# Autodesk Inventor assembly: Pick_&_Place_Nozzle_Assembly
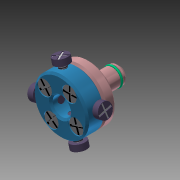
[picture p0: Inventor's stored thumbnail of the model, 180x180]
Saved by Autodesk Inventor 2015 (Build 190159000, 159)
## iProperties
Created: 2015-01-06
Part Number: Pick_&_Place_Nozzle_Assembly
Document SubType Name: Assembly
Designer: ice
Author: ice
## Documents named in this file (8)
- C:\Users\ice\Documents\GitHub\PnP-Magnetic-Tool-Tip\Inventor\Magnetic_Extender_Assembly.iam
- C:\Users\ice\Documents\GitHub\PnP-Magnetic-Tool-Tip\Inventor\Magnet_Extender_Split_Top.ipt
- C:\Users\ice\Documents\GitHub\PnP-Magnetic-Tool-Tip\Inventor\Magnet_Extender_Split_Bottom.ipt
- C:\Users\ice\Documents\GitHub\PnP-Magnetic-Tool-Tip\Inventor\M2x5_D963.ipt
- C:\Users\ice\Documents\GitHub\PnP-Magnetic-Tool-Tip\Inventor\o_ring_3.18_0.5.ipt
- C:\Users\ice\Documents\GitHub\PnP-Magnetic-Tool-Tip\Inventor\M2x5_D85_PANHD.ipt
- C:\Users\ice\Documents\GitHub\PnP-Magnetic-Tool-Tip\Inventor\Magnet10x1x5.ipt
- C:\Users\ice\Documents\GitHub\PnP-Magnetic-Tool-Tip\Inventor\o_ring_4.29_0.5XXX.ipt
## Components (14 placed, 7 different names)
1. Magnet_Extender_Split_Bottom:1 — Mate:2, Mate:4, Mate:5, Mate:6, Mate:7, Mate:8, Mate:9, Mate:10, Mate:11, Mate:14, Mate:15, Mate:16, Mate:17, Mate:19, Flush:1, Mate:20, Flush:2, Mate:22, Mate:23
2. Magnet_Extender_Split_Top:1 — Mate:2, Mate:21, Mate:22, Mate:23, Mate:24, Mate:25, Flush:3, Mate:26, Mate:27, Flush:4, Flush:5, Mate:28, Flush:6
3. M2x5_D963:1 — Mate:4, Mate:5
4. M2x5_D963:2 — Mate:6, Mate:11
5. M2x5_D963:3 — Mate:8, Mate:9
6. M2x5_D963:4 — Mate:7, Mate:10
7. o_ring_3.18_0.5:1 — Mate:24, Mate:25
8. M2x5_D85_PANHD:1 — Mate:16, Flush:2
9. M2x5_D85_PANHD:2 — Mate:15, Mate:20
10. M2x5_D85_PANHD:3 — Mate:14, Mate:19
11. M2x5_D85_PANHD:4 — Mate:17, Flush:1
12. Magnet10x1x5:1 — Mate:21, Flush:3
13. o_ring_4.29_0.5XXX:1 — Mate:27, Flush:4
14. o_ring_4.29_0.5XXX:2 — Mate:26, Flush:5
## Relationships (29: Mate 23, Flush 6)
- Mate:2: Magnet_Extender_Split_Bottom:1 ↔ Magnet_Extender_Split_Top:1
- Mate:4: Magnet_Extender_Split_Bottom:1 ↔ M2x5_D963:1
- Mate:5: Magnet_Extender_Split_Bottom:1 ↔ M2x5_D963:1
- Mate:6: Magnet_Extender_Split_Bottom:1 ↔ M2x5_D963:2
- Mate:7: Magnet_Extender_Split_Bottom:1 ↔ M2x5_D963:4
- Mate:8: Magnet_Extender_Split_Bottom:1 ↔ M2x5_D963:3
- Mate:9: Magnet_Extender_Split_Bottom:1 ↔ M2x5_D963:3
- Mate:10: Magnet_Extender_Split_Bottom:1 ↔ M2x5_D963:4
- Mate:11: Magnet_Extender_Split_Bottom:1 ↔ M2x5_D963:2
- Mate:14: Magnet_Extender_Split_Bottom:1 ↔ M2x5_D85_PANHD:3
- Mate:15: Magnet_Extender_Split_Bottom:1 ↔ M2x5_D85_PANHD:2
- Mate:16: Magnet_Extender_Split_Bottom:1 ↔ M2x5_D85_PANHD:1
- Mate:17: Magnet_Extender_Split_Bottom:1 ↔ M2x5_D85_PANHD:4
- Mate:19: Magnet_Extender_Split_Bottom:1 ↔ M2x5_D85_PANHD:3
- Flush:1: Magnet_Extender_Split_Bottom:1 ↔ M2x5_D85_PANHD:4
- Mate:20: Magnet_Extender_Split_Bottom:1 ↔ M2x5_D85_PANHD:2
- Flush:2: Magnet_Extender_Split_Bottom:1 ↔ M2x5_D85_PANHD:1
- Mate:21: Magnet_Extender_Split_Top:1 ↔ Magnet10x1x5:1
- Mate:22: Magnet_Extender_Split_Bottom:1 ↔ Magnet_Extender_Split_Top:1
- Mate:23: Magnet_Extender_Split_Bottom:1 ↔ Magnet_Extender_Split_Top:1
- Mate:24: Magnet_Extender_Split_Top:1 ↔ o_ring_3.18_0.5:1
- Mate:25: Magnet_Extender_Split_Top:1 ↔ o_ring_3.18_0.5:1
- Flush:3: Magnet_Extender_Split_Top:1 ↔ Magnet10x1x5:1
- Mate:26: Magnet_Extender_Split_Top:1 ↔ o_ring_4.29_0.5XXX:2
- Mate:27: Magnet_Extender_Split_Top:1 ↔ o_ring_4.29_0.5XXX:1
- Flush:4: Magnet_Extender_Split_Top:1 ↔ o_ring_4.29_0.5XXX:1
- Flush:5: Magnet_Extender_Split_Top:1 ↔ o_ring_4.29_0.5XXX:2
- Mate:28: Magnet_Extender_Split_Top:1
- Flush:6: Magnet_Extender_Split_Top:1
